# Autodesk Inventor assembly: Assembly_Cassete_Deck
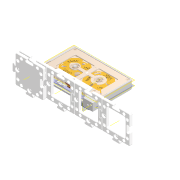
[picture p0: Inventor's stored thumbnail of the model, 180x180]
Saved by Autodesk Inventor 2022 (Build 260153000, 153)
## iProperties
Created: 2023-02-06
Part Number: Assembly_Cassete_Deck
Document SubType Name: Assembly
Designer: diederichbenedict
Author: diederichbenedict
## Documents named in this file (8)
- C:\Users\diederichbenedict\Dropbox\Dokumente\Promotion\PROJECTS\MicroRecord\INVENTOR\Assembly_Cassete_Deck.iam
- C:\Users\diederichbenedict\Dropbox\Dokumente\Promotion\PROJECTS\MicroRecord\INVENTOR\00_Cassette.iam
- C:\Users\diederichbenedict\Dropbox\Dokumente\Promotion\PROJECTS\MicroRecord\INVENTOR\00_Stepper_Motor_28BYJ-48.ipt
- C:\Users\diederichbenedict\Dropbox\Dokumente\Promotion\PROJECTS\MicroRecord\INVENTOR\10_Cassette_microscopy_deck.ipt
- C:\Users\diederichbenedict\Dropbox\Dokumente\Promotion\PROJECTS\MicroRecord\INVENTOR\11_Motor_to_Cassette_Clutch.ipt
- C:\Users\diederichbenedict\Dropbox\Dokumente\Promotion\PROJECTS\MicroRecord\INVENTOR\10_Base_puzzle_v3.ipt
- C:\Users\diederichbenedict\Dropbox\Dokumente\Promotion\PROJECTS\MicroRecord\INVENTOR\10_Cassete_Slide.ipt
- C:\Users\diederichbenedict\Dropbox\Dokumente\Promotion\PROJECTS\MicroRecord\INVENTOR\10_Base_puzzle_cassetteadapter_v3.ipt
## Components (10 placed, 7 different names)
1. 00_Cassette:1 [sub-assembly] — Einfügen:1, Winkel:1, Fluchtend:1, Fluchtend:2, Fluchtend:3, Fluchtend:4, Passend:1
2. 00_Stepper_Motor_28BYJ-48:1 — Einfügen:1, Winkel:1
3. 10_Cassette_microscopy_deck:1 — Fluchtend:1, Fluchtend:2, Passend:2, Winkel:2, Fluchtend:5, Fluchtend:6
4. 11_Motor_to_Cassette_Clutch:1 — Fluchtend:3, Fluchtend:4
5. 10_Cassete_Slide:1 — Fluchtend:5, Fluchtend:6, Passend:3, Winkel:3, Fluchtend:7
6. 10_Base_puzzle_cassetteadapter_v3:1 — Passend:3, Passend:4, Winkel:3, Fluchtend:7
7. 10_Base_puzzle_v3:1 — Passend:1, Passend:2, Winkel:2
8. 10_Base_puzzle_v3:2
9. 10_Base_puzzle_v3:3 — Passend:4
10. 10_Base_puzzle_v3:4
## Component patterns: (4 elements, first: 10_Base_puzzle_v3:1)
## Relationships (15: Flush 7, Mate 4, Angle 3, Insert 1)
- Einfügen:1 [Insert] (-5 mm): 00_Cassette:1 ↔ 00_Stepper_Motor_28BYJ-48:1
- Winkel:1 [Angle] (0 deg): 00_Cassette:1 ↔ 00_Stepper_Motor_28BYJ-48:1
- Fluchtend:1 [Flush]: 00_Cassette:1 ↔ 10_Cassette_microscopy_deck:1
- Fluchtend:2 [Flush]: 00_Cassette:1 ↔ 10_Cassette_microscopy_deck:1
- Fluchtend:3 [Flush]: 00_Cassette:1 ↔ 11_Motor_to_Cassette_Clutch:1
- Fluchtend:4 [Flush]: 00_Cassette:1 ↔ 11_Motor_to_Cassette_Clutch:1
- Passend:1 [Mate]: 00_Cassette:1 ↔ 10_Base_puzzle_v3:1
- Passend:2 [Mate]: 10_Cassette_microscopy_deck:1 ↔ 10_Base_puzzle_v3:1
- Winkel:2 [Angle] (0 deg): 10_Cassette_microscopy_deck:1 ↔ 10_Base_puzzle_v3:1
- Fluchtend:5 [Flush]: 10_Cassette_microscopy_deck:1 ↔ 10_Cassete_Slide:1
- Fluchtend:6 [Flush]: 10_Cassette_microscopy_deck:1 ↔ 10_Cassete_Slide:1
- Passend:3 [Mate]: 10_Cassete_Slide:1 ↔ 10_Base_puzzle_cassetteadapter_v3:1
- Passend:4 [Mate]: 10_Base_puzzle_cassetteadapter_v3:1 ↔ 10_Base_puzzle_v3:3
- Winkel:3 [Angle] (0 deg): 10_Cassete_Slide:1 ↔ 10_Base_puzzle_cassetteadapter_v3:1
- Fluchtend:7 [Flush]: 10_Cassete_Slide:1 ↔ 10_Base_puzzle_cassetteadapter_v3:1
